# Autodesk Inventor assembly: Chessboard Design
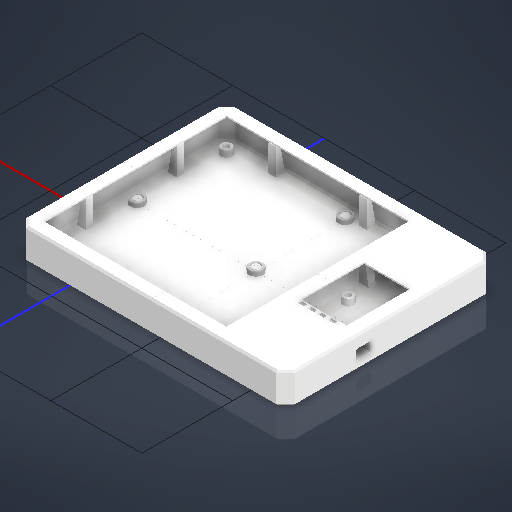
[picture p0: Inventor's stored thumbnail of the model, 512x512]
Saved by Autodesk Inventor 2026 (Build 300175000, 175)
## iProperties
Created: 2025-06-07
Part Number: Chessboard Design
Document SubType Name: Assembly
Designer: ckyiu
Author: ckyiu
## Documents named in this file (3)
- F:\Chessboard-Design\Assemblies\Chessboard Design Case.iam
- F:\Chessboard-Design\Assemblies\Case\Case Bottom.iam
- F:\Chessboard-Design\Assemblies\Case\Case Top.iam
## Components (2 placed, 2 different names)
1. Case Bottom:1 [sub-assembly] — Mate:1, Mate:2, Mate:3
2. Case Top:1 [sub-assembly] — Mate:1, Mate:2, Mate:3
## Relationships (3: Mate 3)
- Mate:1: Case Bottom:1 ↔ Case Top:1
- Mate:2: Case Bottom:1 ↔ Case Top:1
- Mate:3: Case Bottom:1 ↔ Case Top:1
